# Autodesk Inventor assembly: Series Elastic Gearbox
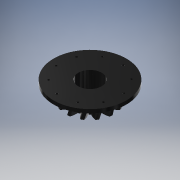
[picture p0: Inventor's stored thumbnail of the model, 180x180]
Saved by Autodesk Inventor 2017 (Build 210142000, 142)
## iProperties
Created: 2019-09-21
Part Number: Series Elastic Gearbox
Document SubType Name: Assembly
Designer: Dell
Author: Dell
## Documents named in this file (5)
- C:\Users\Dell\Documents\GitHub\tr2\Actuator 2.0\Series Elastic Gearbox 1.2\Series Elastic Gearbox 1.2.iam
- C:\Users\Dell\Documents\GitHub\tr2\Actuator 2.0\Series Elastic Gearbox 1.2\SG01.ipt
- C:\Users\Dell\Documents\GitHub\tr2\Actuator 2.0\Series Elastic Gearbox 1.2\SG02.ipt
- C:\Users\Dell\Documents\GitHub\tr2\Actuator 2.0\Series Elastic Gearbox 1.2\SG03.ipt
- C:\Users\Dell\Documents\GitHub\tr2\Actuator 2.0\Series Elastic Gearbox 1.2\SG04.ipt
## Components (4 placed, 4 different names)
1. SG01:1 — Mate:1, Rotation:1, Mate:8, Flush:1, Mate:9
2. SG02:1 — Mate:1, Mate:3, Mate:4, Mate:6, Mate:7, Flush:1
3. SG03:1 — Mate:3, Mate:4, Mate:7, Mate:8
4. Spur Gear1:1 — Mate:6, Rotation:1, Mate:9
## Relationships (9: Mate 7, RelateRotation 1, Flush 1)
- Mate:1: SG01:1 ↔ SG02:1
- Mate:3: SG02:1 ↔ SG03:1
- Mate:4: SG02:1 ↔ SG03:1
- Mate:6: SG02:1 ↔ Spur Gear1:1
- Rotation:1 [RelateRotation] (1 ul): SG01:1 ↔ Spur Gear1:1
- Mate:7: SG02:1 ↔ SG03:1
- Mate:8: SG01:1 ↔ SG03:1
- Flush:1: SG01:1 ↔ SG02:1
- Mate:9: SG01:1 ↔ Spur Gear1:1
